# Autodesk Inventor assembly: Fixation
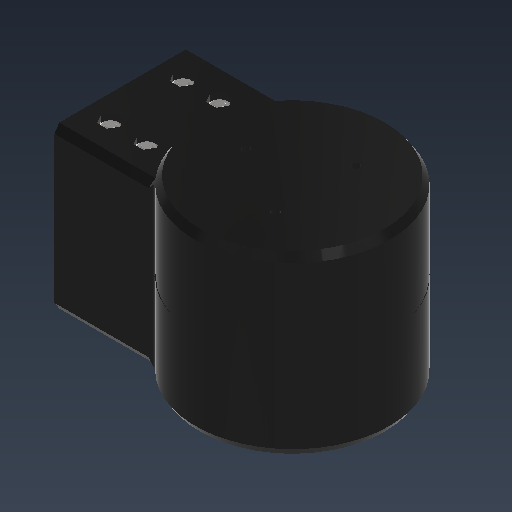
[picture p0: Inventor's stored thumbnail of the model, 512x512]
Saved by Autodesk Inventor 2021 (Build 250183000, 183)
## iProperties
Created: 2025-04-02
Part Number: Fixation
Document SubType Name: Assembly
Designer: rocke
Author: rocke
## Documents named in this file (4)
- C:\Users\rocke\Documents\Robot Arm IPT\Fixation.iam
- C:\Users\rocke\Documents\Robot Arm IPT\Left.ipt
- C:\Users\rocke\Documents\Inventor\Content Center Files\R2021\en-US\ANSI B18.3.1M(1)\ANSI B18.3.1M - M4x0.7 x 60(2).ipt
- C:\Users\rocke\Documents\Inventor\Content Center Files\R2021\en-US\ISO 4032(2)\ISO 4032 - M4 - ISO.ipt
## Components (10 placed, 3 different names)
1. Left:1 — Flush:1, Rigid:1, Mate:1, Mate:2, Mate:3, Mate:4, Mate:5, Mate:6, Mate:7, Mate:8, Mate:9, Mate:11, Mate:13, Mate:15
2. Left:2 — Rigid:1, Mate:10, Mate:12, Mate:14, Mate:16
3. Broached Socket Head Cap Screw - Metric M4x0.7 x 60:1 — Mate:1, Mate:2
4. ISO 4032 M4:1 — Mate:9, Mate:10
5. Broached Socket Head Cap Screw - Metric M4x0.7 x 60:2 — Mate:3, Mate:4
6. Broached Socket Head Cap Screw - Metric M4x0.7 x 60:3 — Mate:5, Mate:6
7. Broached Socket Head Cap Screw - Metric M4x0.7 x 60:4 — Mate:7, Mate:8
8. ISO 4032 M4:2 — Mate:11, Mate:12
9. ISO 4032 M4:3 — Mate:13, Mate:14
10. ISO 4032 M4:4 — Mate:15, Mate:16
## Relationships (18: Mate 16, Flush 1, WeldJoint 1)
- Flush:1: Left:1
- Rigid:1 [WeldJoint]: Left:1 ↔ Left:2
- Mate:1: Left:1 ↔ Broached Socket Head Cap Screw - Metric M4x0.7 x 60:1
- Mate:2: Left:1 ↔ Broached Socket Head Cap Screw - Metric M4x0.7 x 60:1
- Mate:3: Left:1 ↔ Broached Socket Head Cap Screw - Metric M4x0.7 x 60:2
- Mate:4: Left:1 ↔ Broached Socket Head Cap Screw - Metric M4x0.7 x 60:2
- Mate:5: Left:1 ↔ Broached Socket Head Cap Screw - Metric M4x0.7 x 60:3
- Mate:6: Left:1 ↔ Broached Socket Head Cap Screw - Metric M4x0.7 x 60:3
- Mate:7: Left:1 ↔ Broached Socket Head Cap Screw - Metric M4x0.7 x 60:4
- Mate:8: Left:1 ↔ Broached Socket Head Cap Screw - Metric M4x0.7 x 60:4
- Mate:9: Left:1 ↔ ISO 4032 M4:1
- Mate:10: Left:2 ↔ ISO 4032 M4:1
- Mate:11: Left:1 ↔ ISO 4032 M4:2
- Mate:12: Left:2 ↔ ISO 4032 M4:2
- Mate:13: Left:1 ↔ ISO 4032 M4:3
- Mate:14: Left:2 ↔ ISO 4032 M4:3
- Mate:15: Left:1 ↔ ISO 4032 M4:4
- Mate:16: Left:2 ↔ ISO 4032 M4:4
